# Autodesk Inventor assembly: Chest
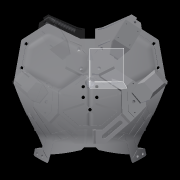
[picture p0: Inventor's stored thumbnail of the model, 180x180]
Saved by Autodesk Inventor 2015 SP1 (Build 190203100, 203)
## iProperties
Created: 2015-04-21
Part Number: Chest
Document SubType Name: Assembly
Designer: Val
Author: Val
## Documents named in this file (4)
- E:\Exo\Models\3D\Chest.iam
- E:\Exo\Models\3D\ChestBase.ipt
- E:\Exo\Models\3D\ChestPlateRight.ipt
- E:\Exo\Models\3D\ChestPlateLeft.ipt
## Components (3 placed, 3 different names)
1. ChestBase:1 — Mate:3
2. ChestPlateRight:1 — Flush:1, Flush:2, Mate:2, Mate:3
3. ChestPlateLeft:1 — Flush:1, Flush:2, Mate:2
## Relationships (4: Flush 2, Mate 2)
- Flush:1: ChestPlateRight:1 ↔ ChestPlateLeft:1
- Flush:2: ChestPlateRight:1 ↔ ChestPlateLeft:1
- Mate:2 (18 mm): ChestPlateRight:1 ↔ ChestPlateLeft:1
- Mate:3: ChestBase:1 ↔ ChestPlateRight:1
